# Autodesk Inventor assembly: mainASM
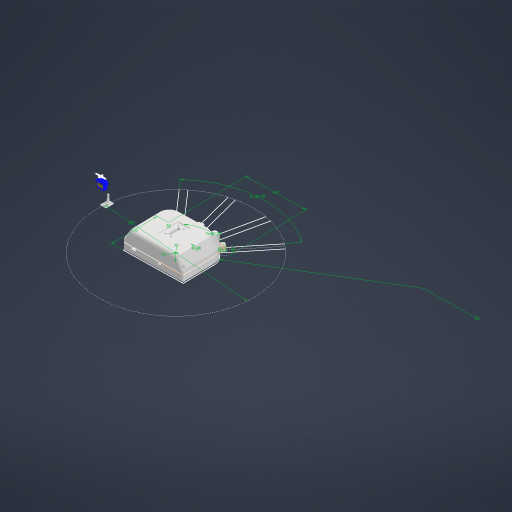
[picture p0: Inventor's stored thumbnail of the model, 512x512]
Saved by Autodesk Inventor 2024 (Build 280153000, 153)
## iProperties
Created: 2024-03-11
Part Number: mainASM
Document SubType Name: Assembly
Designer: Daniel
Author: Daniel
## Documents named in this file (8)
- C:\Users\Daniel\Desktop\pmik_2024l_jd\mechanical\mainASM.iam
- C:\Users\Daniel\Desktop\pmik_2024l_jd\mechanical\STEPS\NUCLEO-F091RC.iam
- C:\Users\Daniel\Desktop\pmik_2024l_jd\mechanical\STEPS\SG90 - Micro Servo 9g - Tower Pro.iam
- C:\Users\Daniel\Desktop\pmik_2024l_jd\mechanical\STEPS\KY-040 Rotary Encoder.iam
- C:\Users\Daniel\Desktop\pmik_2024l_jd\mechanical\bottom.ipt
- C:\Users\Daniel\Desktop\pmik_2024l_jd\mechanical\Pump.ipt
- C:\Users\Daniel\Desktop\pmik_2024l_jd\mechanical\STEPS\LM2596 DC to DC Buck Converter 3 A.iam
- C:\Users\Daniel\Desktop\pmik_2024l_jd\mechanical\Top.ipt
## Components (7 placed, 7 different names)
1. NUCLEO-F091RC:1 [sub-assembly] — Mate:3, Mate:4, Mate:5
2. SG90 - Micro Servo 9g - Tower Pro:1 [sub-assembly]
3. KY-040 Rotary Encoder:1 [sub-assembly]
4. bottom:1 — Flush:1, Angle:1, Mate:3, Mate:4, Mate:5, Mate:6, Mate:7, Mate:8, Mate:9, Flush:2, Flush:3, Flush:4, Flush:5
5. Pump:1 — Angle:1, Mate:6, Mate:7, Mate:8
6. LM2596 DC to DC Buck Converter 3 A:1 [sub-assembly] — Mate:9, Flush:2, Flush:3
7. Top:1 — Flush:4, Flush:5
## Relationships (13: Mate 7, Flush 5, Angle 1)
- Flush:1: bottom:1
- Angle:1 (180 deg): bottom:1 ↔ Pump:1
- Mate:3 (3 mm): NUCLEO-F091RC:1 ↔ bottom:1
- Mate:4 (2 mm): NUCLEO-F091RC:1 ↔ bottom:1
- Mate:5 (5 mm): NUCLEO-F091RC:1 ↔ bottom:1
- Mate:6 (25 mm): bottom:1 ↔ Pump:1
- Mate:7 (5 mm): bottom:1 ↔ Pump:1
- Mate:8 (3 mm): bottom:1 ↔ Pump:1
- Mate:9 (5 mm): bottom:1 ↔ LM2596 DC to DC Buck Converter 3 A:1
- Flush:2 (5 mm): bottom:1 ↔ LM2596 DC to DC Buck Converter 3 A:1
- Flush:3 (4 mm): bottom:1 ↔ LM2596 DC to DC Buck Converter 3 A:1
- Flush:4: bottom:1 ↔ Top:1
- Flush:5: bottom:1 ↔ Top:1
